# Autodesk Inventor assembly: Energy_Pack
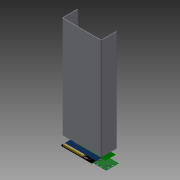
[picture p0: Inventor's stored thumbnail of the model, 180x180]
Saved by Autodesk Inventor 2016 (Build 200138000, 138)
## iProperties
Created: 2015-03-25
Part Number: Energy_Pack
Document SubType Name: Assembly
Designer: Yann
Author: Yann
## Documents named in this file (6)
- C:\Users\Yann\Documents\GitHub\Bikair_CAD\Source\Energy_Pack\Energy_Pack.iam
- C:\Users\Yann\Documents\GitHub\Bikair_CAD\Source\Energy_Pack\Casing.iam
- C:\Users\Yann\Documents\GitHub\Bikair_CAD\Source\Energy_Pack\PCB_Altium_Exports\Backbone.ipt
- C:\Users\Yann\Documents\GitHub\Bikair_CAD\Source\Energy_Pack\PCB_Altium_Exports\BMS.ipt
- C:\Users\Yann\Documents\GitHub\Bikair_CAD\Source\Energy_Pack\PCB_Altium_Exports\Buck_Boost_PFC.ipt
- C:\Users\Yann\Documents\GitHub\Bikair_CAD\Source\Energy_Pack\PCB_Altium_Exports\Power_PCB.ipt
## Components (5 placed, 5 different names)
1. Casing:1 [sub-assembly] — Affleurement:1, Affleurement:2, Affleurement:3, Flush:4
2. Backbone:1 — Rigid:1
3. BMS:1
4. Buck_Boost_PFC:1 — Flush:5
5. Power_PCB:1 — Flush:4, Rigid:1, Flush:5
## Relationships (6: Flush 5, WeldJoint 1)
- Affleurement:1 [Flush]: Casing:1
- Affleurement:2 [Flush]: Casing:1
- Affleurement:3 [Flush]: Casing:1
- Flush:4 (-50 mm): Casing:1 ↔ Power_PCB:1
- Rigid:1 [WeldJoint]: Backbone:1 ↔ Power_PCB:1
- Flush:5: Buck_Boost_PFC:1 ↔ Power_PCB:1
